# Autodesk Inventor assembly: Prensa_Hidraulica
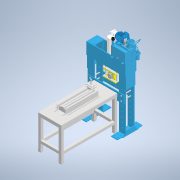
[picture p0: Inventor's stored thumbnail of the model, 180x180]
Saved by Autodesk Inventor 2021 (Build 250183000, 183)
## iProperties
Created: 2020-01-15
Part Number: Prensa_Hidraulica
Document SubType Name: Assembly
Designer: Nelson
Sending System: SolidWorks 2020
Last Author: Micro
Last Saved: 2020-01-16
Author: Nelson
## Documents named in this file (12)
- D:\Nelson\Documentos\Inventor\PrensaHidraulica_Automatizada\Prensa_Hidraulica.iam
- Prensa_Hidraulica.iam
- D:\Nelson\Documentos\Inventor\PrensaHidraulica_Automatizada\Estructura.iam
- D:\Nelson\Documentos\Inventor\PrensaHidraulica_Automatizada\Cilindro neumatico.ipt
- D:\Nelson\Documentos\Inventor\PrensaHidraulica_Automatizada\Bomba Hidraulica.ipt
- D:\Nelson\Documentos\Inventor\PrensaHidraulica_Automatizada\Ensamble Mecanismo cilindro.iam
- D:\Nelson\Documentos\Inventor\PrensaHidraulica_Automatizada\PH 013.ipt
- D:\Nelson\Documentos\Inventor\PrensaHidraulica_Automatizada\Mesa.iam
- D:\Nelson\Documentos\Inventor\PrensaHidraulica_Automatizada\Barra_5-8_950.ipt
- D:\Nelson\Documentos\Inventor\PrensaHidraulica_Automatizada\PerfilZ.ipt
- D:\Nelson\Documentos\Inventor\PrensaHidraulica_Automatizada\Angulo en V.ipt
- D:\Nelson\Documentos\Inventor\PrensaHidraulica_Automatizada\TUBING NOTCHER DIE.iam
## Components (15 placed, 10 different names)
1. Cilindro neumatico:1 — Mate:2, Mate:3, Mate:52
2. Bomba Hidraulica:1 — Mate:1, Flush:1, Flush:2
3. PH 013:3 — Mate:40, Mate:42
4. PH 013:4 — Mate:41, Mate:43
5. PH 013:5 — Mate:34, Mate:35
6. PH 013:6 — Mate:32, Mate:33
7. Ensamble mecanismo cilindro:1 [sub-assembly] — Tangent:1, Tangent:2, Mate:46, Flush:4, Mate:49, Mate:50, Flush:5
8. Mesa:1 [sub-assembly] — Mate:44, Mate:45, Mate:46, Flush:4, Mate:47, Mate:48, Flush:6, Flush:7, Flush:8
9. Barra_5-8_950:1 — Tangent:1, Tangent:2, Flush:5
10. PerfilZ:1 — Mate:47, Mate:49
11. PerfilZ:2 — Mate:48, Mate:50
12. Angulo en V:1 — Flush:6
13. Angulo en V:2 — Flush:7
14. TUBING NOTCHER DIE:1 [sub-assembly] — Mate:52
15. Estructura:1 [sub-assembly] — Mate:1, Flush:1, Flush:2, Mate:2, Mate:3, Mate:32, Mate:33, Mate:34, Mate:35, Mate:40, Mate:41, Mate:42, Mate:43, Mate:44, Mate:45, Flush:8
## Relationships (28: Mate 19, Flush 7, Tangent 2)
- Mate:1: Bomba Hidraulica:1 ↔ Estructura:1
- Flush:1: Bomba Hidraulica:1 ↔ Estructura:1
- Flush:2: Bomba Hidraulica:1 ↔ Estructura:1
- Mate:2: Cilindro neumatico:1 ↔ Estructura:1
- Mate:3: Cilindro neumatico:1 ↔ Estructura:1
- Mate:32: PH 013:6 ↔ Estructura:1
- Mate:33: PH 013:6 ↔ Estructura:1
- Mate:34: PH 013:5 ↔ Estructura:1
- Mate:35: PH 013:5 ↔ Estructura:1
- Mate:40: PH 013:3 ↔ Estructura:1
- Mate:41: PH 013:4 ↔ Estructura:1
- Mate:42: PH 013:3 ↔ Estructura:1
- Mate:43: PH 013:4 ↔ Estructura:1
- Mate:44: Mesa:1 ↔ Estructura:1
- Mate:45 (25 mm): Mesa:1 ↔ Estructura:1
- Tangent:1: Ensamble mecanismo cilindro:1 ↔ Barra_5-8_950:1
- Tangent:2: Ensamble mecanismo cilindro:1 ↔ Barra_5-8_950:1
- Mate:46: Ensamble mecanismo cilindro:1 ↔ Mesa:1
- Flush:4 (275 mm): Ensamble mecanismo cilindro:1 ↔ Mesa:1
- Mate:47: Mesa:1 ↔ PerfilZ:1
- Mate:48: Mesa:1 ↔ PerfilZ:2
- Mate:49: Ensamble mecanismo cilindro:1 ↔ PerfilZ:1
- Mate:50: Ensamble mecanismo cilindro:1 ↔ PerfilZ:2
- Flush:5 (-50 mm): Ensamble mecanismo cilindro:1 ↔ Barra_5-8_950:1
- Flush:6: Mesa:1 ↔ Angulo en V:1
- Flush:7: Mesa:1 ↔ Angulo en V:2
- Mate:52: Cilindro neumatico:1 ↔ TUBING NOTCHER DIE:1
- Flush:8: Mesa:1 ↔ Estructura:1
